# Autodesk Inventor assembly: Grabber Tool
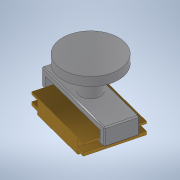
[picture p0: Inventor's stored thumbnail of the model, 180x180]
Saved by Autodesk Inventor 2022 (Build 260153000, 153)
## iProperties
Created: 2020-12-03
Part Number: Grabber Tool
Document SubType Name: Assembly
Designer: caleb
Author: caleb
## Documents named in this file (5)
- C:\Users\Caleb\Desktop\nebraska-silicon-lab\Hardware\ETL\Module Assembly\Grabber Tool - V2\Grabber Tool - V2.iam
- C:\Users\Caleb\Desktop\nebraska-silicon-lab\Hardware\ETL\Module Assembly\Grabber Tool - V2\Grabber Base - V2.ipt
- C:\Users\Caleb\Desktop\nebraska-silicon-lab\Hardware\ETL\Module Assembly\Grabber Tool - V2\Grabber Platform - V2.ipt
- C:\Users\Caleb\Desktop\nebraska-silicon-lab\Hardware\ETL\Module Assembly\Grabber Tool - V2\92125A130_TYPE 18-8 SS FLAT-HEAD SOCKET CAP SCREW.ipt
- C:\Users\Caleb\Desktop\nebraska-silicon-lab\Hardware\ETL\Module Assembly\Glue Stamp - V2\Stamp Assembly - V2.iam
## Components (7 placed, 4 different names)
1. Grabber Base - V2:1 — Insert:1, Insert:2
2. Grabber Platform - V2:1 — Insert:1, Insert:2, Mate:1, Mate:2, Mate:3, Mate:4, Mate:5, Angle:1
3. 92125A130_TYPE 18-8 SS FLAT-HEAD SOCKET CAP SCREW:1 — Mate:2
4. 92125A130_TYPE 18-8 SS FLAT-HEAD SOCKET CAP SCREW:2 — Mate:1
5. 92125A130_TYPE 18-8 SS FLAT-HEAD SOCKET CAP SCREW:3 — Mate:4
6. 92125A130_TYPE 18-8 SS FLAT-HEAD SOCKET CAP SCREW:4 — Mate:3
7. Stamp Assembly - V2:1 [sub-assembly] — Mate:5, Angle:1
## Relationships (8: Mate 5, Insert 2, Angle 1)
- Insert:1: Grabber Base - V2:1 ↔ Grabber Platform - V2:1
- Insert:2: Grabber Base - V2:1 ↔ Grabber Platform - V2:1
- Mate:1: Grabber Platform - V2:1 ↔ 92125A130_TYPE 18-8 SS FLAT-HEAD SOCKET CAP SCREW:2
- Mate:2: Grabber Platform - V2:1 ↔ 92125A130_TYPE 18-8 SS FLAT-HEAD SOCKET CAP SCREW:1
- Mate:3: Grabber Platform - V2:1 ↔ 92125A130_TYPE 18-8 SS FLAT-HEAD SOCKET CAP SCREW:4
- Mate:4: Grabber Platform - V2:1 ↔ 92125A130_TYPE 18-8 SS FLAT-HEAD SOCKET CAP SCREW:3
- Mate:5: Grabber Platform - V2:1 ↔ Stamp Assembly - V2:1
- Angle:1 (0 deg): Grabber Platform - V2:1 ↔ Stamp Assembly - V2:1
